# Autodesk Inventor assembly: Chassis 2012
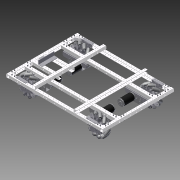
[picture p0: Inventor's stored thumbnail of the model, 180x180]
Saved by Autodesk Inventor 2012 SP1 (Build 160190100, 190)
## iProperties
Created: 2012-01-19
Part Number: Chassis 2012
Document SubType Name: Assembly
Designer: cheehan jeremy
Mass: 25347.6 g
Surface Area: 39867.6 cm^2
Volume: 16865.8 cm^3
Density: 1.5029 g/cm^3
Author: cheehan jeremy
## Documents named in this file (41)
- K:\MHS\Technology\Holliday B\Group Projects\Robotics\CAD Team\CAD Team 2013\Chassis\Full Chassis\Chassis 2012.iam
- Chassis 2012.iam
- K:\MHS\Technology\Holliday B\Group Projects\Robotics\CAD Team\2012 Robot\Chassis\8 Mecanum Right\8 Inch Mecanum Right.iam
- K:\MHS\Technology\Holliday B\Group Projects\Robotics\CAD Team\2012 Robot\Final Sub-Assemblies\Ball.ipt
- K:\MHS\Technology\Holliday B\Group Projects\Robotics\CAD Team\CAD Team 2013\Chassis\Full Chassis\Chassis_Base.iam
- K:\MHS\Technology\Holliday B\Group Projects\Robotics\CAD Team\2012 Robot\Chassis\Toughbox\Toughbox Nano.iam
- K:\MHS\Technology\Holliday B\Group Projects\Robotics\CAD Team\2012 Robot\Chassis\8 Mecanum Left\8 Inch Mecanum Left.iam
- K:\MHS\Technology\Holliday B\Group Projects\Robotics\CAD Team\2012 Robot\Ball Pickup\Roller.ipt
- K:\MHS\Technology\Holliday B\Group Projects\Robotics\CAD Team\2012 Robot\Chassis\Toughbox\GearBox Bracket.ipt
- K:\MHS\Technology\Holliday B\Group Projects\Robotics\CAD Team\2012 Robot\Chassis\Toughbox\Toughbox Bracket.ipt
- K:\MHS\Technology\Holliday B\Group Projects\Robotics\CAD Team\2012 Robot\Chassis\Toughbox\Toughbox Bracket Mirrored.ipt
- K:\MHS\Technology\Holliday B\Group Projects\Robotics\CAD Team\2012 Robot\Chassis\Toughbox\Bearing Bracket.ipt
- K:\MHS\Technology\Holliday B\Group Projects\Robotics\CAD Team\2012 Robot\Chassis\Toughbox\Bearing Bracket 2.ipt
- K:\MHS\Technology\Holliday B\Group Projects\Robotics\CAD Team\2012 Robot\Chassis\Toughbox\Hub.ipt
- K:\MHS\Technology\Holliday B\Group Projects\Robotics\CAD Team\2012 Robot\Chassis\Chassis 2012A\Design Accelerator\Bolted Connection3.iam
- K:\MHS\Technology\Holliday B\Group Projects\Robotics\CAD Team\2012 Robot\Chassis\Chassis 2012A\Design Accelerator\Bolted Connection5.iam
- K:\MHS\Technology\Holliday B\Group Projects\Robotics\CAD Team\2012 Robot\Chassis\Chassis 2012A\Design Accelerator\Bolted Connection6.iam
- K:\MHS\Technology\Holliday B\Group Projects\Robotics\CAD Team\2012 Robot\Chassis\Chassis 2012A\Design Accelerator\Bolted Connection7.iam
- K:\MHS\Technology\Holliday B\Group Projects\Robotics\CAD Team\2012 Robot\Chassis\Chassis 2012A\Design Accelerator\Bolted Connection8.iam
- K:\MHS\Technology\Holliday B\Group Projects\Robotics\CAD Team\2012 Robot\Chassis\Chassis 2012A\Design Accelerator\Bolted Connection9.iam
- K:\MHS\Technology\Holliday B\Group Projects\Robotics\CAD Team\2012 Robot\Chassis\Chassis 2012A\Design Accelerator\Bolted Connection10.iam
- K:\MHS\Technology\Holliday B\Group Projects\Robotics\CAD Team\2012 Robot\Chassis\Chassis 2012A\Design Accelerator\Bolted Connection11.iam
- K:\MHS\Technology\Holliday B\Group Projects\Robotics\CAD Team\2012 Robot\Chassis\Chassis 2012A\Design Accelerator\Bolted Connection12.iam
- K:\MHS\Technology\Holliday B\Group Projects\Robotics\CAD Team\2012 Robot\Chassis\Chassis 2012A\Design Accelerator\Bolted Connection13.iam
- K:\MHS\Technology\Holliday B\Group Projects\Robotics\CAD Team\2012 Robot\Chassis\Chassis 2012A\Design Accelerator\Bolted Connection14.iam
- K:\MHS\Technology\Holliday B\Group Projects\Robotics\CAD Team\2012 Robot\Chassis\Chassis 2012A\Design Accelerator\Bolted Connection15.iam
- K:\MHS\Technology\Holliday B\Group Projects\Robotics\CAD Team\2012 Robot\Chassis\Chassis 2012A\Design Accelerator\Bolted Connection16.iam
- K:\MHS\Technology\Holliday B\Group Projects\Robotics\CAD Team\2012 Robot\Chassis\Chassis 2012A\Design Accelerator\Bolted Connection17.iam
- K:\MHS\Technology\Holliday B\Group Projects\Robotics\CAD Team\2012 Robot\Chassis\Chassis 2012A\Design Accelerator\Bolted Connection1.iam
- K:\MHS\Technology\Holliday B\Group Projects\Robotics\CAD Team\2012 Robot\Chassis\Chassis 2012A\Design Accelerator\Bolted Connection2.iam
- K:\MHS\Technology\Holliday B\Group Projects\Robotics\CAD Team\2012 Robot\Chassis\Chassis 2012A\Design Accelerator\Bolted Connection4.iam
- K:\MHS\Technology\Holliday B\Group Projects\Robotics\CAD Team\2012 Robot\Chassis\Chassis 2012A\Design Accelerator\Bolted Connection18.iam
- K:\MHS\Technology\Holliday B\Group Projects\Robotics\CAD Team\2012 Robot\Chassis\Chassis 2012A\Design Accelerator\Bolted Connection19.iam
- K:\MHS\Technology\Holliday B\Group Projects\Robotics\CAD Team\2012 Robot\Chassis\Chassis 2012A\Design Accelerator\Bolted Connection20.iam
- K:\MHS\Technology\Holliday B\Group Projects\Robotics\CAD Team\2012 Robot\Chassis\Chassis 2012\Design Accelerator\Bolted Connection1.iam
- K:\MHS\Technology\Holliday B\Group Projects\Robotics\CAD Team\2012 Robot\Chassis\Frame\Chassis_Channel_10_AndyMark_am-0202.ipt
- K:\MHS\Technology\Holliday B\Group Projects\Robotics\CAD Team\2012 Robot\Chassis\Frame\Chassis_CornerConnect_AndyMark_am-0212.ipt
- K:\MHS\Technology\Holliday B\Group Projects\Robotics\CAD Team\2012 Robot\Final Sub-Assemblies\Chassis 2012\Design Accelerator\Bolted Connection1.iam
- K:\MHS\Technology\Holliday B\Group Projects\Robotics\CAD Team\2012 Robot\Final Sub-Assemblies\Chassis 2012\Design Accelerator\Bolted Connection2.iam
- K:\MHS\Technology\Holliday B\Group Projects\Robotics\CAD Team\2012 Robot\Electrical\Battery Mount.ipt
- K:\MHS\Technology\Holliday B\Group Projects\Robotics\CAD Team\2012 Robot\Final Sub-Assemblies\Chassis 2012\Design Accelerator\Bolted Connection3.iam
## Components (63 placed, 16 different names)
1. Chassis_Base:1 [sub-assembly] — Flush:10, Flush:11, Flush:12, Flush:13, Tangent:4, Flush:14, Tangent:5, Flush:15, Tangent:6, Tangent:7, Insert:1, Insert:2, Insert:3, Insert:4, Insert:7, Insert:8, Insert:9, Insert:10, Insert:15, Insert:16, Insert:21, Insert:22, Insert:24, Insert:25, Mate:66, Mate:67, Insert:26, Insert:27, Mate:70, Mate:71, Mate:72, Mate:73, Insert:28, Insert:29, Insert:30, Insert:31, Mate:78, Mate:79, Mate:86, Flush:31, Mate:88, Insert:37, Mate:89, Insert:38, Insert:40, Insert:42, Mate:92, Mate:93, Mate:94, Mate:97, Mate:98, Mate:99, Mate:100, Mate:102, Mate:103
2. Toughbox Nano:6 [sub-assembly] — Mate:21, Flush:29, Mate:22, Mate:24
3. Toughbox Nano:3 [sub-assembly] — Mate:15, Flush:25, Mate:17, Mate:26
4. Toughbox Nano:4 [sub-assembly] — Angle:2, Mate:8, Flush:19, Mate:18, Flush:27, Mate:20, Mate:25
5. Toughbox Nano:5 [sub-assembly] — Mate:10, Angle:4, Flush:20, Mate:11, Mate:12, Flush:23, Mate:14
6. 8 Inch Mecanum Left:2 [sub-assembly]
7. 8 Inch Mecanum Right:2 [sub-assembly] — Angle:2, Mate:8, Flush:19
8. Ball:1 — Tangent:1
9. Ball:2 — Tangent:2
10. 8 Inch Mecanum Left:1 [sub-assembly] — Mate:10, Angle:4, Flush:20
11. 8 Inch Mecanum Right:3 [sub-assembly]
12. Roller:1 — Tangent:3, Flush:13, Tangent:4
13. Roller:2 — Flush:15, Tangent:6, Tangent:7
14. Roller:3 — Flush:14, Mate:6, Tangent:5
15. GearBox Bracket:1 — Mate:23, Flush:30, Mate:24, Insert:3, Insert:4
16. GearBox Bracket:2 — Mate:16, Flush:26, Mate:17, Insert:24, Insert:25, Mate:74, Mate:75
17. GearBox Bracket:3 — Mate:19, Flush:28, Mate:20, Insert:1, Insert:2, Mate:76, Mate:77
18. GearBox Bracket:4 — Mate:13, Mate:14, Flush:24, Insert:26, Insert:27
19. Toughbox Bracket:1 — Mate:11, Mate:12, Flush:23, Mate:13, Flush:24
20. Toughbox Bracket:2 — Mate:21, Flush:29, Mate:22, Mate:23, Flush:30
21. Toughbox Bracket Mirrored:1 — Mate:15, Flush:25, Mate:16, Flush:26, Mate:26
22. Toughbox Bracket Mirrored:2 — Mate:18, Flush:27, Mate:19, Flush:28, Mate:25
23. Bearing Bracket:1 — Insert:19, Insert:20, Mate:27, Mate:28, Tangent:8, Mate:42, Mate:43, Mate:44, Mate:45
24. Bearing Bracket:2 — Insert:17, Insert:18, Mate:30, Mate:31, Tangent:9, Mate:38, Mate:39, Mate:40, Mate:41
25. Bearing Bracket:3 — Insert:11, Insert:12, Mate:34, Mate:35, Tangent:11
26. Bearing Bracket:4 — Insert:5, Insert:6, Mate:32, Mate:33, Tangent:10
27. Bearing Bracket 2:1 — Insert:5, Insert:6, Insert:7, Insert:8, Mate:50, Mate:51, Mate:52, Mate:53
28. Bearing Bracket 2:2 — Insert:15, Insert:16, Insert:17, Insert:18
29. Bearing Bracket 2:3 — Insert:9, Insert:10, Insert:11, Insert:12, Mate:46, Mate:47, Mate:48, Mate:49, Mate:82, Mate:83
30. Bearing Bracket 2:4 — Insert:19, Insert:20, Insert:21, Insert:22, Insert:23
31. Hub:1 — Mate:32, Mate:33, Tangent:10, Mate:60, Mate:61, Insert:33
32. Hub:2 — Mate:27, Mate:29, Tangent:8, Mate:62, Mate:63
33. Hub:3 — Mate:34, Mate:35, Mate:56, Mate:57, Mate:58, Mate:59, Insert:34, Mate:84, Mate:85
34. Hub:4 — Mate:30, Mate:31, Tangent:9, Insert:32
35. Bolted Connection:1 [sub-assembly] — Insert:23, Mate:82, Mate:83
36. Bolted Connection:2 [sub-assembly] — Mate:38, Mate:39
37. Bolted Connection:3 [sub-assembly] — Mate:40, Mate:41
38. Bolted Connection:4 [sub-assembly] — Mate:42, Mate:43
39. Bolted Connection:5 [sub-assembly] — Mate:44, Mate:45
40. Bolted Connection:6 [sub-assembly] — Mate:46, Mate:47
41. Bolted Connection:7 [sub-assembly] — Mate:48, Mate:49
42. Bolted Connection:8 [sub-assembly] — Mate:50, Mate:51
43. Bolted Connection:9 [sub-assembly] — Mate:52, Mate:53
44. Bolted Connection:10 [sub-assembly] — Mate:84, Mate:85
45. Bolted Connection:11 [sub-assembly] — Mate:56, Mate:57, Tangent:11
46. Bolted Connection:12 [sub-assembly] — Mate:58, Mate:59, Insert:34
47. Bolted Connection:13 [sub-assembly] — Mate:60, Mate:61, Insert:33
48. Bolted Connection:14 [sub-assembly] — Mate:62, Mate:63, Insert:32
49. Bolted Connection:15 [sub-assembly] — Insert:30, Mate:99, Mate:100
50. Bolted Connection:16 [sub-assembly] — Mate:66, Mate:67, Insert:31
51. Bolted Connection:17 [sub-assembly] — Mate:70, Mate:71, Insert:28
52. Bolted Connection:18 [sub-assembly] — Mate:72, Mate:73, Insert:29
53. Bolted Connection:19 [sub-assembly] — Mate:74, Mate:75
54. Bolted Connection:20 [sub-assembly] — Mate:76, Mate:77
55. Bolted Connection:21 [sub-assembly] — Mate:78, Mate:79
56. Chassis_Channel_10_AndyMark_am-0202:1 — Mate:86, Flush:31, Insert:37, Insert:39, Mate:96
57. Chassis_Channel_10_AndyMark_am-0202:2 — Mate:88, Mate:89, Insert:38, Insert:41, Mate:101, Flush:32
58. Chassis_CornerConnect_AndyMark_am-0212:1 — Insert:39, Insert:40
59. Chassis_CornerConnect_AndyMark_am-0212:2 — Insert:41, Insert:42
60. Bolted Connection:22 [sub-assembly] — Mate:96, Mate:97, Mate:98, Tangent:12
61. Bolted Connection:23 [sub-assembly] — Mate:92, Mate:93, Mate:94
62. Battery Mount:1 — Mate:101, Flush:32, Tangent:12
63. Bolted Connection:24 [sub-assembly] — Mate:102, Mate:103
## Relationships (159: Mate 85, Insert 38, Flush 20, Tangent 12, Angle 4)
- Angle:2 (0 deg): Toughbox Nano:4 ↔ 8 Inch Mecanum Right:2
- Flush:10 (139.7 mm): Chassis_Base:1
- Tangent:1: Ball:1
- Tangent:2: Ball:2
- Flush:11: Chassis_Base:1
- Mate:5
- Flush:12: Chassis_Base:1
- Tangent:3 (190.5 mm): Roller:1
- Flush:13 (266.7 mm): Chassis_Base:1 ↔ Roller:1
- Tangent:4: Chassis_Base:1 ↔ Roller:1
- Flush:14 (266.7 mm): Chassis_Base:1 ↔ Roller:3
- Mate:6 (-381 mm): Roller:3
- Tangent:5: Chassis_Base:1 ↔ Roller:3
- Flush:15 (266.7 mm): Chassis_Base:1 ↔ Roller:2
- Tangent:6 (121.2334 mm): Chassis_Base:1 ↔ Roller:2
- Tangent:7 (121.2334 mm): Chassis_Base:1 ↔ Roller:2
- [Mate]: Toughbox Nano:6 ↔ 8 Inch Mecanum Left:2
- Mate:8: Toughbox Nano:4 ↔ 8 Inch Mecanum Right:2
- [Mate]: Toughbox Nano:3 ↔ 8 Inch Mecanum Right:3
- Mate:10: Toughbox Nano:5 ↔ 8 Inch Mecanum Left:1
- Angle:4 (180 deg): Toughbox Nano:5 ↔ 8 Inch Mecanum Left:1
- [Angle] (180 deg): Toughbox Nano:3 ↔ 8 Inch Mecanum Right:3
- [Angle] (180 deg): Toughbox Nano:6 ↔ 8 Inch Mecanum Left:2
- Flush:19 (-19.05 mm): Toughbox Nano:4 ↔ 8 Inch Mecanum Right:2
- Flush:20 (-19.05 mm): Toughbox Nano:5 ↔ 8 Inch Mecanum Left:1
- [Flush] (19.05 mm): Toughbox Nano:3 ↔ 8 Inch Mecanum Right:3
- [Flush] (19.05 mm): Toughbox Nano:6 ↔ 8 Inch Mecanum Left:2
- Mate:11: Toughbox Nano:5 ↔ Toughbox Bracket:1
- Mate:12: Toughbox Nano:5 ↔ Toughbox Bracket:1
- Flush:23 (-44.45 mm): Toughbox Nano:5 ↔ Toughbox Bracket:1
- Mate:13: GearBox Bracket:4 ↔ Toughbox Bracket:1
- Mate:14: Toughbox Nano:5 ↔ GearBox Bracket:4
- Flush:24: GearBox Bracket:4 ↔ Toughbox Bracket:1
- Mate:15: Toughbox Nano:3 ↔ Toughbox Bracket Mirrored:1
- Flush:25 (-44.45 mm): Toughbox Nano:3 ↔ Toughbox Bracket Mirrored:1
- Mate:16: GearBox Bracket:2 ↔ Toughbox Bracket Mirrored:1
- Flush:26: GearBox Bracket:2 ↔ Toughbox Bracket Mirrored:1
- Mate:17: Toughbox Nano:3 ↔ GearBox Bracket:2
- Mate:18: Toughbox Nano:4 ↔ Toughbox Bracket Mirrored:2
- Flush:27 (-44.45 mm): Toughbox Nano:4 ↔ Toughbox Bracket Mirrored:2
- Mate:19: GearBox Bracket:3 ↔ Toughbox Bracket Mirrored:2
- Flush:28: GearBox Bracket:3 ↔ Toughbox Bracket Mirrored:2
- Mate:20: Toughbox Nano:4 ↔ GearBox Bracket:3
- Mate:21: Toughbox Nano:6 ↔ Toughbox Bracket:2
- Flush:29 (-44.45 mm): Toughbox Nano:6 ↔ Toughbox Bracket:2
- Mate:22: Toughbox Nano:6 ↔ Toughbox Bracket:2
- Mate:23: GearBox Bracket:1 ↔ Toughbox Bracket:2
- Flush:30: GearBox Bracket:1 ↔ Toughbox Bracket:2
- Mate:24: Toughbox Nano:6 ↔ GearBox Bracket:1
- Mate:25: Toughbox Nano:4 ↔ Toughbox Bracket Mirrored:2
- Insert:1: Chassis_Base:1 ↔ GearBox Bracket:3
- Insert:2: Chassis_Base:1 ↔ GearBox Bracket:3
- Insert:3: Chassis_Base:1 ↔ GearBox Bracket:1
- Insert:4: Chassis_Base:1 ↔ GearBox Bracket:1
- Insert:5: Bearing Bracket:4 ↔ Bearing Bracket 2:1
- Insert:6: Bearing Bracket:4 ↔ Bearing Bracket 2:1
- Insert:7: Chassis_Base:1 ↔ Bearing Bracket 2:1
- Insert:8: Chassis_Base:1 ↔ Bearing Bracket 2:1
- Insert:9: Chassis_Base:1 ↔ Bearing Bracket 2:3
- Insert:10: Chassis_Base:1 ↔ Bearing Bracket 2:3
- Insert:11: Bearing Bracket:3 ↔ Bearing Bracket 2:3
- Insert:12: Bearing Bracket:3 ↔ Bearing Bracket 2:3
- Insert:15: Chassis_Base:1 ↔ Bearing Bracket 2:2
- Insert:16: Chassis_Base:1 ↔ Bearing Bracket 2:2
- Insert:17: Bearing Bracket:2 ↔ Bearing Bracket 2:2
- Insert:18: Bearing Bracket:2 ↔ Bearing Bracket 2:2
- Insert:19: Bearing Bracket:1 ↔ Bearing Bracket 2:4
- Insert:20: Bearing Bracket:1 ↔ Bearing Bracket 2:4
- Mate:26: Toughbox Nano:3 ↔ Toughbox Bracket Mirrored:1
- Mate:27: Bearing Bracket:1 ↔ Hub:2
- Mate:28: Bearing Bracket:1
- Mate:29: Hub:2
- Tangent:8: Bearing Bracket:1 ↔ Hub:2
- Mate:30: Bearing Bracket:2 ↔ Hub:4
- Mate:31: Bearing Bracket:2 ↔ Hub:4
- Tangent:9: Bearing Bracket:2 ↔ Hub:4
- Mate:32: Bearing Bracket:4 ↔ Hub:1
- Mate:33: Bearing Bracket:4 ↔ Hub:1
- Tangent:10: Bearing Bracket:4 ↔ Hub:1
- Mate:34: Bearing Bracket:3 ↔ Hub:3
- Mate:35: Bearing Bracket:3 ↔ Hub:3
- Mate:38: Bearing Bracket:2 ↔ Bolted Connection:2
- Mate:39: Bearing Bracket:2 ↔ Bolted Connection:2
- Mate:40: Bearing Bracket:2 ↔ Bolted Connection:3
- Mate:41: Bearing Bracket:2 ↔ Bolted Connection:3
- Mate:42: Bearing Bracket:1 ↔ Bolted Connection:4
- Mate:43: Bearing Bracket:1 ↔ Bolted Connection:4
- Mate:44: Bearing Bracket:1 ↔ Bolted Connection:5
- Mate:45: Bearing Bracket:1 ↔ Bolted Connection:5
- Mate:46: Bearing Bracket 2:3 ↔ Bolted Connection:6
- Mate:47: Bearing Bracket 2:3 ↔ Bolted Connection:6
- Mate:48: Bearing Bracket 2:3 ↔ Bolted Connection:7
- Mate:49: Bearing Bracket 2:3 ↔ Bolted Connection:7
- Mate:50: Bearing Bracket 2:1 ↔ Bolted Connection:8
- Mate:51: Bearing Bracket 2:1 ↔ Bolted Connection:8
- Mate:52: Bearing Bracket 2:1 ↔ Bolted Connection:9
- Mate:53: Bearing Bracket 2:1 ↔ Bolted Connection:9
- Mate:56: Hub:3 ↔ Bolted Connection:11
- Mate:57: Hub:3 ↔ Bolted Connection:11
- Mate:58: Hub:3 ↔ Bolted Connection:12
- Mate:59: Hub:3 ↔ Bolted Connection:12
- Mate:60: Hub:1 ↔ Bolted Connection:13
- Mate:61: Hub:1 ↔ Bolted Connection:13
- Mate:62: Hub:2 ↔ Bolted Connection:14
- Mate:63: Hub:2 ↔ Bolted Connection:14
- Insert:21: Chassis_Base:1 ↔ Bearing Bracket 2:4
- Insert:22: Chassis_Base:1 ↔ Bearing Bracket 2:4
- Insert:23: Bearing Bracket 2:4 ↔ Bolted Connection:1
- Insert:24: Chassis_Base:1 ↔ GearBox Bracket:2
- Insert:25: Chassis_Base:1 ↔ GearBox Bracket:2
- Mate:66: Chassis_Base:1 ↔ Bolted Connection:16
- Mate:67: Chassis_Base:1 ↔ Bolted Connection:16
- Insert:26: Chassis_Base:1 ↔ GearBox Bracket:4
- Insert:27: Chassis_Base:1 ↔ GearBox Bracket:4
- Mate:70: Chassis_Base:1 ↔ Bolted Connection:17
- Mate:71: Chassis_Base:1 ↔ Bolted Connection:17
- Mate:72: Chassis_Base:1 ↔ Bolted Connection:18
- Mate:73: Chassis_Base:1 ↔ Bolted Connection:18
- Mate:74: GearBox Bracket:2 ↔ Bolted Connection:19
- Mate:75: GearBox Bracket:2 ↔ Bolted Connection:19
- Mate:76: GearBox Bracket:3 ↔ Bolted Connection:20
- Mate:77: GearBox Bracket:3 ↔ Bolted Connection:20
- Insert:28: Chassis_Base:1 ↔ Bolted Connection:17
- Insert:29: Chassis_Base:1 ↔ Bolted Connection:18
- Insert:30: Chassis_Base:1 ↔ Bolted Connection:15
- Insert:31: Chassis_Base:1 ↔ Bolted Connection:16
- Insert:32: Hub:4 ↔ Bolted Connection:14
- Insert:33: Hub:1 ↔ Bolted Connection:13
- Insert:34: Hub:3 ↔ Bolted Connection:12
- Mate:78: Chassis_Base:1 ↔ Bolted Connection:21
- Mate:79: Chassis_Base:1 ↔ Bolted Connection:21
- Tangent:11: Bearing Bracket:3 ↔ Bolted Connection:11
- Mate:82: Bearing Bracket 2:3 ↔ Bolted Connection:1
- Mate:83: Bearing Bracket 2:3 ↔ Bolted Connection:1
- Mate:84: Hub:3 ↔ Bolted Connection:10
- Mate:85: Hub:3 ↔ Bolted Connection:10
- Mate:86: Chassis_Base:1 ↔ Chassis_Channel_10_AndyMark_am-0202:1
- Flush:31: Chassis_Base:1 ↔ Chassis_Channel_10_AndyMark_am-0202:1
- Mate:88: Chassis_Base:1 ↔ Chassis_Channel_10_AndyMark_am-0202:2
- Insert:37: Chassis_Base:1 ↔ Chassis_Channel_10_AndyMark_am-0202:1
- Mate:89: Chassis_Base:1 ↔ Chassis_Channel_10_AndyMark_am-0202:2
- Insert:38: Chassis_Base:1 ↔ Chassis_Channel_10_AndyMark_am-0202:2
- Insert:39: Chassis_Channel_10_AndyMark_am-0202:1 ↔ Chassis_CornerConnect_AndyMark_am-0212:1
- Insert:40: Chassis_Base:1 ↔ Chassis_CornerConnect_AndyMark_am-0212:1
- Insert:41: Chassis_Channel_10_AndyMark_am-0202:2 ↔ Chassis_CornerConnect_AndyMark_am-0212:2
- Insert:42: Chassis_Base:1 ↔ Chassis_CornerConnect_AndyMark_am-0212:2
- Mate:92: Chassis_Base:1 ↔ Bolted Connection:23
- Mate:93: Chassis_Base:1 ↔ Bolted Connection:23
- Mate:94: Chassis_Base:1 ↔ Bolted Connection:23
- Mate:96: Chassis_Channel_10_AndyMark_am-0202:1 ↔ Bolted Connection:22
- Mate:97: Chassis_Base:1 ↔ Bolted Connection:22
- Mate:98: Chassis_Base:1 ↔ Bolted Connection:22
- Mate:99: Chassis_Base:1 ↔ Bolted Connection:15
- Mate:100: Chassis_Base:1 ↔ Bolted Connection:15
- Mate:101: Chassis_Channel_10_AndyMark_am-0202:2 ↔ Battery Mount:1
- Flush:32 (3.175 mm): Chassis_Channel_10_AndyMark_am-0202:2 ↔ Battery Mount:1
- Tangent:12 (1.5875 mm): Bolted Connection:22 ↔ Battery Mount:1
- Mate:102: Chassis_Base:1 ↔ Bolted Connection:24
- Mate:103: Chassis_Base:1 ↔ Bolted Connection:24
